# Autodesk Inventor assembly: default_motor_asembly
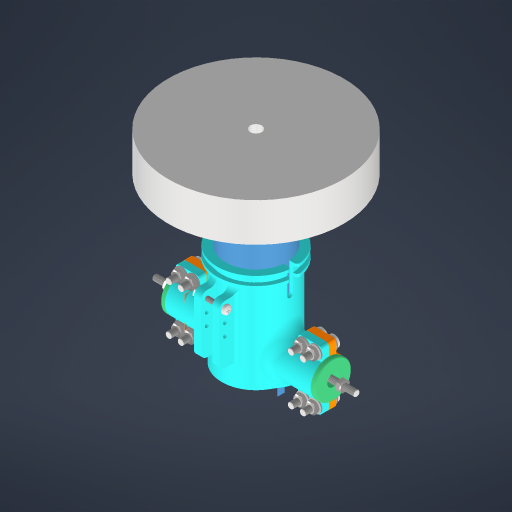
[picture p0: Inventor's stored thumbnail of the model, 512x512]
Saved by Autodesk Inventor 2024 (Build 280153000, 153)
## iProperties
Created: 2023-05-13
Part Number: default_motor_asembly
Document SubType Name: Assembly
Designer: user
Mass: 558.582 g
Surface Area: 1019.17 cm^2
Volume: 517.598 cm^3
Density: 1.07918 g/cm^3
Author: user
## Documents named in this file (11)
- D:\Docs\Robot\3d\motor_assembly\default_motor_asembly.iam
- D:\Docs\Robot\3d\motor_assembly\default_motor_asembly\lower_arm.ipt
- D:\Docs\Robot\3d\motor_assembly\bushing_assembly.iam
- D:\Docs\Robot\3d\default_components\motor.ipt
- C:\Users\user\Documents\Inventor\Content Center Files\R2024\ru-RU\DIN 125-1  A\DIN 125 - A 4,3.ipt
- C:\Users\user\Documents\Inventor\Content Center Files\R2024\ru-RU\DIN 7985 (H)\DIN 7985 (H) - M4x20-H.ipt
- C:\Users\user\Documents\Inventor\Content Center Files\R2024\ru-RU\DIN 934\DIN 934 - M4 x 0,7.ipt
- D:\Docs\Robot\3d\default_components\wheel.ipt
- D:\Docs\Robot\3d\motor_assembly\default_motor_asembly\cup.ipt
- C:\Users\user\Documents\Inventor\Content Center Files\R2024\ru-RU\DIN 7985 (H)\DIN 7985 (H) - M3x20-H.ipt
- C:\Users\user\Documents\Inventor\Content Center Files\R2024\ru-RU\DIN 934\DIN 934 - M3 x 0,5.ipt
## Components (41 placed, 10 different names)
1. lower_arm:1 — Совмещение:1, Совмещение:2, Совмещение:3, Вставка:2, Вставка:6, Совмещение:4, Вставка:7, Вставка:8, Вставка:13, Вставка:14, Вставка:15, Вставка:16, Заподлицо:1, Заподлицо:3, Вставка:28, Вставка:29, Вставка:48, Вставка:49, Вставка:50
2. bushing_assembly:1 [sub-assembly] — Заподлицо:2, Заподлицо:3
3. bushing_assembly:2 [sub-assembly] — Вставка:2
4. motor:1 — Вставка:23, Вставка:50
5. DIN 125-1 A A 4,3:1 — Вставка:6, Вставка:41
6. DIN 125-1 A A 4,3:2 — Совмещение:4, Вставка:45
7. DIN 125-1 A A 4,3:3 — Вставка:8, Вставка:47
8. DIN 125-1 A A 4,3:4 — Вставка:7, Вставка:46
9. DIN 125-1 A A 4,3:5 — Вставка:24, Вставка:44
10. DIN 125-1 A A 4,3:6 — Вставка:26, Вставка:42
11. DIN 125-1 A A 4,3:7 — Вставка:27, Вставка:40
12. DIN 125-1 A A 4,3:8 — Вставка:25, Вставка:43
13. DIN 125-1 A A 4,3:9 — Вставка:13, Вставка:22
14. DIN 125-1 A A 4,3:10 — Вставка:14, Вставка:39
15. DIN 125-1 A A 4,3:11 — Вставка:15, Вставка:38
16. DIN 125-1 A A 4,3:12 — Вставка:16, Вставка:37
17. DIN 125-1 A A 4,3:13 — Вставка:30, Вставка:35
18. DIN 125-1 A A 4,3:14 — Вставка:31, Вставка:34
19. DIN 125-1 A A 4,3:15 — Вставка:32, Вставка:36
20. DIN 125-1 A A 4,3:16 — Вставка:21, Вставка:33
21. DIN 7985 (H) M4x20-H:1 — Вставка:21
22. DIN 934 - заменено на DIN EN 24032/28673/28674 M4:1 — Вставка:22
23. wheel:1 — Вставка:23
24. cup:1 — Заподлицо:1, Заподлицо:2, Вставка:24, Вставка:25, Вставка:26, Вставка:27
25. cup:2 — Вставка:28, Вставка:29, Вставка:30, Вставка:31, Вставка:32, Вставка:33
26. DIN 7985 (H) M4x20-H:2 — Вставка:40
27. DIN 934 - заменено на DIN EN 24032/28673/28674 M4:2 — Вставка:41
28. DIN 7985 (H) M4x20-H:3 — Вставка:36
29. DIN 934 - заменено на DIN EN 24032/28673/28674 M4:3 — Вставка:37
30. DIN 7985 (H) M4x20-H:4 — Вставка:35
31. DIN 934 - заменено на DIN EN 24032/28673/28674 M4:4 — Вставка:38
32. DIN 7985 (H) M4x20-H:5 — Вставка:34
33. DIN 934 - заменено на DIN EN 24032/28673/28674 M4:5 — Вставка:39
34. DIN 7985 (H) M4x20-H:6 — Вставка:44
35. DIN 7985 (H) M4x20-H:7 — Вставка:43
36. DIN 7985 (H) M4x20-H:8 — Вставка:42
37. DIN 934 - заменено на DIN EN 24032/28673/28674 M4:6 — Вставка:45
38. DIN 934 - заменено на DIN EN 24032/28673/28674 M4:7 — Вставка:46
39. DIN 934 - заменено на DIN EN 24032/28673/28674 M4:8 — Вставка:47
40. DIN 7985 (H) M3x20-H:4 — Вставка:48
41. DIN 934 - заменено на DIN EN 24032/28673/28674 M3:1 — Вставка:49
## Relationships (45: Insert 38, Mate 4, Flush 3)
- Совмещение:1 [Mate]: lower_arm:1
- Совмещение:2 [Mate]: lower_arm:1
- Совмещение:3 [Mate]: lower_arm:1
- Вставка:2 [Insert]: lower_arm:1 ↔ bushing_assembly:2
- Вставка:6 [Insert]: lower_arm:1 ↔ DIN 125-1 A A 4,3:1
- Совмещение:4 [Mate]: lower_arm:1 ↔ DIN 125-1 A A 4,3:2
- Вставка:7 [Insert]: lower_arm:1 ↔ DIN 125-1 A A 4,3:4
- Вставка:8 [Insert]: lower_arm:1 ↔ DIN 125-1 A A 4,3:3
- Вставка:13 [Insert]: lower_arm:1 ↔ DIN 125-1 A A 4,3:9
- Вставка:14 [Insert]: lower_arm:1 ↔ DIN 125-1 A A 4,3:10
- Вставка:15 [Insert]: lower_arm:1 ↔ DIN 125-1 A A 4,3:11
- Вставка:16 [Insert]: lower_arm:1 ↔ DIN 125-1 A A 4,3:12
- Вставка:21 [Insert]: DIN 125-1 A A 4,3:16 ↔ DIN 7985 (H) M4x20-H:1
- Вставка:22 [Insert]: DIN 125-1 A A 4,3:9 ↔ DIN 934 - заменено на DIN EN 24032/28673/28674 M4:1
- Вставка:23 [Insert]: motor:1 ↔ wheel:1
- Заподлицо:1 [Flush]: lower_arm:1 ↔ cup:1
- Заподлицо:2 [Flush]: bushing_assembly:1 ↔ cup:1
- Вставка:24 [Insert]: DIN 125-1 A A 4,3:5 ↔ cup:1
- Вставка:25 [Insert]: DIN 125-1 A A 4,3:8 ↔ cup:1
- Вставка:26 [Insert]: DIN 125-1 A A 4,3:6 ↔ cup:1
- Вставка:27 [Insert]: DIN 125-1 A A 4,3:7 ↔ cup:1
- Заподлицо:3 [Flush]: lower_arm:1 ↔ bushing_assembly:1
- Вставка:28 [Insert]: lower_arm:1 ↔ cup:2
- Вставка:29 [Insert]: lower_arm:1 ↔ cup:2
- Вставка:30 [Insert]: DIN 125-1 A A 4,3:13 ↔ cup:2
- Вставка:31 [Insert]: DIN 125-1 A A 4,3:14 ↔ cup:2
- Вставка:32 [Insert]: DIN 125-1 A A 4,3:15 ↔ cup:2
- Вставка:33 [Insert]: DIN 125-1 A A 4,3:16 ↔ cup:2
- Вставка:34 [Insert]: DIN 125-1 A A 4,3:14 ↔ DIN 7985 (H) M4x20-H:5
- Вставка:35 [Insert]: DIN 125-1 A A 4,3:13 ↔ DIN 7985 (H) M4x20-H:4
- Вставка:36 [Insert]: DIN 125-1 A A 4,3:15 ↔ DIN 7985 (H) M4x20-H:3
- Вставка:37 [Insert]: DIN 125-1 A A 4,3:12 ↔ DIN 934 - заменено на DIN EN 24032/28673/28674 M4:3
- Вставка:38 [Insert]: DIN 125-1 A A 4,3:11 ↔ DIN 934 - заменено на DIN EN 24032/28673/28674 M4:4
- Вставка:39 [Insert]: DIN 125-1 A A 4,3:10 ↔ DIN 934 - заменено на DIN EN 24032/28673/28674 M4:5
- Вставка:40 [Insert]: DIN 125-1 A A 4,3:7 ↔ DIN 7985 (H) M4x20-H:2
- Вставка:41 [Insert]: DIN 125-1 A A 4,3:1 ↔ DIN 934 - заменено на DIN EN 24032/28673/28674 M4:2
- Вставка:42 [Insert]: DIN 125-1 A A 4,3:6 ↔ DIN 7985 (H) M4x20-H:8
- Вставка:43 [Insert]: DIN 125-1 A A 4,3:8 ↔ DIN 7985 (H) M4x20-H:7
- Вставка:44 [Insert]: DIN 125-1 A A 4,3:5 ↔ DIN 7985 (H) M4x20-H:6
- Вставка:45 [Insert]: DIN 125-1 A A 4,3:2 ↔ DIN 934 - заменено на DIN EN 24032/28673/28674 M4:6
- Вставка:46 [Insert]: DIN 125-1 A A 4,3:4 ↔ DIN 934 - заменено на DIN EN 24032/28673/28674 M4:7
- Вставка:47 [Insert]: DIN 125-1 A A 4,3:3 ↔ DIN 934 - заменено на DIN EN 24032/28673/28674 M4:8
- Вставка:48 [Insert]: lower_arm:1 ↔ DIN 7985 (H) M3x20-H:4
- Вставка:49 [Insert]: lower_arm:1 ↔ DIN 934 - заменено на DIN EN 24032/28673/28674 M3:1
- Вставка:50 [Insert]: lower_arm:1 ↔ motor:1
